# Autodesk Inventor assembly: PILLARSCELLCASE21700ASSEMBLY
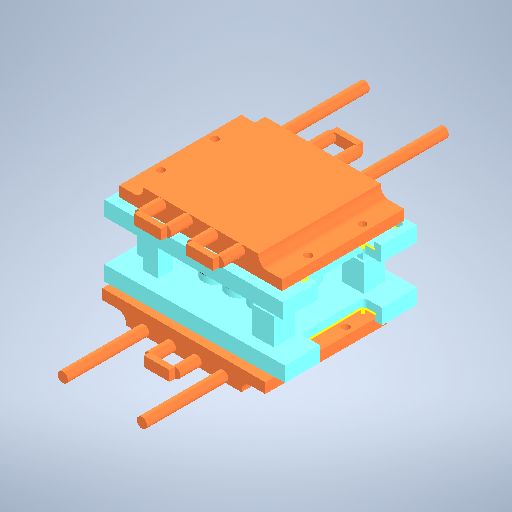
[picture p0: Inventor's stored thumbnail of the model, 512x512]
Saved by Autodesk Inventor 2025.2 (Build 292293000, 293)
## iProperties
Created: 2025-06-10
Part Number: PILLARSCELLCASE21700ASSEMBLY
Document SubType Name: Assembly
Designer: cbast
Author: cbast
## Documents named in this file (5)
- C:\Users\cbast\OneDrive\Documents\GitHub\Smart-Pack-for-Advanced-Research-and-Control\variations\Camden\V0.2\PILLARSCELLCASE21700ASSEMBLY.iam
- C:\Users\cbast\OneDrive\Documents\GitHub\Smart-Pack-for-Advanced-Research-and-Control\variations\Camden\V0.1\21700(Blue).ipt
- C:\Users\cbast\OneDrive\Documents\GitHub\Smart-Pack-for-Advanced-Research-and-Control\variations\Camden\V0.1\343thermalpad.ipt
- C:\Users\cbast\OneDrive\Documents\GitHub\Smart-Pack-for-Advanced-Research-and-Control\variations\Camden\V0.1\cooling plate.ipt
- C:\Users\cbast\OneDrive\Documents\GitHub\Smart-Pack-for-Advanced-Research-and-Control\variations\Camden\V0.2\PILLARSCELLCASE21700.ipt
## Components (7 placed, 4 different names)
1. 21700(Blue):1 — Mate:1, Mate:2, Mate:5, Mate:8
2. 343thermalpad:1 — Mate:2, Mate:3
3. 343thermalpad:2 — Mate:1, Mate:4
4. cooling plate:1 — Mate:3
5. cooling plate:2 — Mate:4, Mate:6, Mate:7
6. PILLARSCELLCASE21700:1 — Mate:5, Mate:6, Mate:7, Mate:9
7. PILLARSCELLCASE21700:2 — Mate:8, Mate:9
## Relationships (9: Mate 9)
- Mate:1: 21700(Blue):1 ↔ 343thermalpad:2
- Mate:2: 21700(Blue):1 ↔ 343thermalpad:1
- Mate:3: 343thermalpad:1 ↔ cooling plate:1
- Mate:4: 343thermalpad:2 ↔ cooling plate:2
- Mate:5: 21700(Blue):1 ↔ PILLARSCELLCASE21700:1
- Mate:6: cooling plate:2 ↔ PILLARSCELLCASE21700:1
- Mate:7: cooling plate:2 ↔ PILLARSCELLCASE21700:1
- Mate:8: 21700(Blue):1 ↔ PILLARSCELLCASE21700:2
- Mate:9: PILLARSCELLCASE21700:1 ↔ PILLARSCELLCASE21700:2
